# Autodesk Inventor assembly: CyberOrto
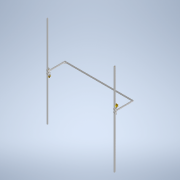
[picture p0: Inventor's stored thumbnail of the model, 180x180]
Saved by Autodesk Inventor 2022 (Build 260153000, 153)
## iProperties
RuleStatus: InUse
Created: 2021-12-29
Part Number: CyberOrto
Document SubType Name: Assembly
Designer: matte
Author: matte
## Documents named in this file (26)
- C:\Users\Elia\Documents\ELIA\UNITN\MAGISTRALE\1st year\1st semester\Mechanical Design\MDM-CyberOrto-CAD\CyberOrto.iam
- C:\Users\Elia\Documents\ELIA\UNITN\MAGISTRALE\1st year\1st semester\Mechanical Design\MDM-CyberOrto-CAD\Pezzi singoli\Trave Principale.ipt
- C:\Users\Elia\Documents\ELIA\UNITN\MAGISTRALE\1st year\1st semester\Mechanical Design\MDM-CyberOrto-CAD\Pezzi singoli\Supporto SX.ipt
- C:\Users\Elia\Documents\ELIA\UNITN\MAGISTRALE\1st year\1st semester\Mechanical Design\MDM-CyberOrto-CAD\Parker components\03-Brackets_Gussets_Plates\09-Machined Gussets\20-102.ipt
- C:\Users\Elia\Documents\ELIA\UNITN\MAGISTRALE\1st year\1st semester\Mechanical Design\MDM-CyberOrto-CAD\Parker components\02-Fasteners\10-Standard T-Nuts\20-050.ipt
- C:\Users\Elia\Documents\ELIA\UNITN\MAGISTRALE\1st year\1st semester\Mechanical Design\MDM-CyberOrto-CAD\Parker components\02-Fasteners\16-Screws\01-Metric Screws\01-Button Head\24-118-8.ipt
- C:\Users\Elia\Documents\ELIA\UNITN\MAGISTRALE\1st year\1st semester\Mechanical Design\MDM-CyberOrto-CAD\Guida a terra.iam
- C:\Users\Elia\Documents\ELIA\UNITN\MAGISTRALE\1st year\1st semester\Mechanical Design\MDM-CyberOrto-CAD\Parker components\05-Handles_Hinges\13-Pivot Joints\23-010.iam
- C:\Users\Elia\Documents\ELIA\UNITN\MAGISTRALE\1st year\1st semester\Mechanical Design\MDM-CyberOrto-CAD\Parker components\02-Fasteners\10-Standard T-Nuts\20-058.ipt
- C:\Users\Elia\Documents\ELIA\UNITN\MAGISTRALE\1st year\1st semester\Mechanical Design\MDM-CyberOrto-CAD\Parker components\02-Fasteners\16-Screws\01-Metric Screws\01-Button Head\24-116-8.ipt
- C:\Users\Elia\Documents\ELIA\UNITN\MAGISTRALE\1st year\1st semester\Mechanical Design\MDM-CyberOrto-CAD\Pezzi singoli\Supporto DX.ipt
- C:\Users\Elia\Documents\ELIA\UNITN\MAGISTRALE\1st year\1st semester\Mechanical Design\MDM-CyberOrto-CAD\Parker components\02-Fasteners\16-Screws\01-Metric Screws\01-Button Head\24-120-8.ipt
- C:\Users\Elia\Documents\ELIA\UNITN\MAGISTRALE\1st year\1st semester\Mechanical Design\MDM-CyberOrto-CAD\Pezzi singoli\Supporto lineare\Carrello semplice.iam
- C:\Users\Elia\Documents\ELIA\UNITN\MAGISTRALE\1st year\1st semester\Mechanical Design\MDM-CyberOrto-CAD\Platform.ipt
- C:\Users\Elia\Documents\ELIA\UNITN\MAGISTRALE\1st year\1st semester\Mechanical Design\MDM-CyberOrto-CAD\Parker components\02-Fasteners\16-Screws\01-Metric Screws\01-Button Head\24-130-6.ipt
- C:\Users\Elia\Documents\ELIA\UNITN\MAGISTRALE\1st year\1st semester\Mechanical Design\MDM-CyberOrto-CAD\Parker components\02-Fasteners\15-T-Bolts_Nuts_Washers\03-Washers\24-700-6.ipt
- C:\Users\Elia\Documents\ELIA\UNITN\MAGISTRALE\1st year\1st semester\Mechanical Design\MDM-CyberOrto-CAD\Parker components\02-Fasteners\15-T-Bolts_Nuts_Washers\02-Nuts\24-706-6.ipt
- C:\Users\Elia\Documents\ELIA\UNITN\MAGISTRALE\1st year\1st semester\Mechanical Design\MDM-CyberOrto-CAD\Servo Motor 50W\bch2mba531ca5c.ipt
- C:\Users\Elia\Documents\ELIA\UNITN\MAGISTRALE\1st year\1st semester\Mechanical Design\MDM-CyberOrto-CAD\Rack_Pinion\Rack gear scaled1.ipt
- C:\Users\Elia\Documents\ELIA\UNITN\MAGISTRALE\1st year\1st semester\Mechanical Design\MDM-CyberOrto-CAD\Rack_Pinion\pinion_scaled1.ipt
- C:\Users\Elia\Documents\ELIA\UNITN\MAGISTRALE\1st year\1st semester\Mechanical Design\MDM-CyberOrto-CAD\Inventor Support\Content Center Files\it-IT\ISO 1580\ISO 1580 - M4 x 12_.ipt
- C:\Users\Elia\Documents\ELIA\UNITN\MAGISTRALE\1st year\1st semester\Mechanical Design\MDM-CyberOrto-CAD\Inventor Support\Content Center Files\it-IT\AS 1474(1)\AS 1474 - M4(1).ipt
- C:\Users\Elia\Documents\ELIA\UNITN\MAGISTRALE\1st year\1st semester\Mechanical Design\MDM-CyberOrto-CAD\Trave a terra\Trave a terra.iam
- C:\Users\Elia\Documents\ELIA\UNITN\MAGISTRALE\1st year\1st semester\Mechanical Design\MDM-CyberOrto-CAD\Racks.iam
- C:\Users\Elia\Documents\ELIA\UNITN\MAGISTRALE\1st year\1st semester\Mechanical Design\MDM-CyberOrto-CAD\Parker components\02-Fasteners\16-Screws\01-Metric Screws\03-Socket Head\24-320-8SS.ipt
- C:\Users\Elia\Documents\ELIA\UNITN\MAGISTRALE\1st year\1st semester\Mechanical Design\MDM-CyberOrto-CAD\Parker components\02-Fasteners\10-Standard T-Nuts\20-058SS.ipt
## Components (86 placed, 25 different names)
1. Trave Principale:1 — Coincidente:1, Coincidente:2, Coincidente:3, Allineato:1, Coincidente:4, Allineato:2, Coincidente:5, Coincidente:10, Coincidente:40, Allineato:5, Allineato:6, Coincidente:41, Angolo:1
2. Supporto SX:1 — Allineato:1, Coincidente:4, Allineato:2, Coincidente:6, Allineato:3, Coincidente:7, Coincidente:15, Coincidente:16, Coincidente:23, Coincidente:28, Coincidente:29, Coincidente:30
3. Supporto DX:1 — Coincidente:45, Allineato:7, Allineato:8, Coincidente:48, Allineato:9, Allineato:10
4. Trave a terra:1 [sub-assembly] — Angolo:2, Angolo:3, Angolo:4, Allineato:59, Coincidente:130, Coincidente:169, Angolo:5, Coincidente:171, Allineato:62, Allineato:88, Coincidente:187, Coincidente:189
5. 20-058SS:1 — Coincidente:186, Coincidente:187
6. 20-058SS:2 — Coincidente:188, Coincidente:189
7. 24-118-8:3 — Coincidente:19, Coincidente:20
8. 24-118-8:4 — Coincidente:21, Coincidente:22
9. 20-050:2 — Coincidente:10, Coincidente:11, Coincidente:12
10. 24-118-8:1 — Coincidente:13, Coincidente:14
11. 24-118-8:2 — Coincidente:17, Coincidente:18
12. 20-102:1 — Coincidente:5, Coincidente:6, Allineato:3, Coincidente:8, Coincidente:9, Coincidente:11, Coincidente:12, Coincidente:13, Coincidente:14, Coincidente:17, Coincidente:18, Coincidente:19, Coincidente:20, Coincidente:21, Coincidente:22
13. 20-050:1 — Coincidente:7, Coincidente:8, Coincidente:9
14. 24-118-8:5 — Coincidente:31, Coincidente:32, Coincidente:33
15. 24-118-8:6 — Coincidente:34, Coincidente:35
16. 24-118-8:7 — Coincidente:38, Coincidente:39
17. 24-118-8:8 — Coincidente:36, Coincidente:37
18. Guida a terra:1 [sub-assembly] — Coincidente:15, Coincidente:16, Coincidente:23, Coincidente:32, Coincidente:33, Coincidente:34, Coincidente:35, Coincidente:36, Coincidente:37, Coincidente:38, Coincidente:39, Coincidente:138, Coincidente:139, Allineato:61, Coincidente:141, Coincidente:143, Coincidente:145, Coincidente:162
19. 20-050:3 — Coincidente:27, Allineato:4, Coincidente:28, Coincidente:30, Coincidente:31
20. 20-050:4 — Coincidente:27, Allineato:4, Coincidente:29
21. 23-010:1 [sub-assembly] — Coincidente:40, Allineato:5, Allineato:6, Coincidente:43, Coincidente:44, Coincidente:45, Allineato:7, Allineato:8, Coincidente:46, Coincidente:47
22. 20-058:1 — Coincidente:41, Angolo:1, Coincidente:42
23. 24-116-8:1 — Coincidente:42, Coincidente:43, Coincidente:44
24. 24-120-8:1 — Coincidente:46, Coincidente:47
25. 24-120-8:2 — Coincidente:51, Coincidente:52
26. Carrello semplice:1 [sub-assembly] — Coincidente:48, Allineato:9, Allineato:10, Coincidente:51, Coincidente:52, Coincidente:53, Allineato:13, Coincidente:54, Coincidente:56, Coincidente:58, Coincidente:60, Coincidente:62, Angolo:2, Angolo:3, Angolo:4, Allineato:59, Coincidente:130
27. 24-130-6:1 — Inserimento:1, Coincidente:61
28. 24-700-6:1 — Inserimento:1, Inserimento:7
29. 24-706-6:1 — Coincidente:55, Coincidente:56
30. 24-130-6:2 — Coincidente:59
31. 24-700-6:3 — Inserimento:6
32. 24-130-6:3 — Coincidente:57
33. 24-700-6:2 — Inserimento:8
34. 24-130-6:4 — Coincidente:55
35. 24-700-6:4 — Inserimento:5
36. 24-706-6:2 — Coincidente:57, Coincidente:58
37. 24-706-6:3 — Coincidente:61, Coincidente:62
38. 24-706-6:4 — Coincidente:59, Coincidente:60
39. Platform:1 — Coincidente:53, Allineato:13, Coincidente:54, Inserimento:5, Inserimento:6, Inserimento:7, Inserimento:8, Coincidente:63, Coincidente:64, Coincidente:65, Coincidente:66, Coincidente:67, Coincidente:68, Coincidente:114, Coincidente:117, Coincidente:121, Coincidente:125, Coincidente:129
40. ISO 1580 M4 x 12:2 — Coincidente:126, Coincidente:127, Coincidente:128
41. AS 1474 - Metrico M4:2 — Coincidente:120, Coincidente:121
42. AS 1474 - Metrico M4:3 — Coincidente:124, Coincidente:125
43. AS 1474 - Metrico M4:4 — Coincidente:128, Coincidente:129
44. ISO 1580 M4 x 12:4 — Coincidente:118, Coincidente:119, Coincidente:120
45. ISO 1580 M4 x 12:3 — Coincidente:122, Coincidente:123, Coincidente:124
46. AS 1474 - Metrico M4:1 — Coincidente:116, Coincidente:117
47. ISO 1580 M4 x 12:1 — Coincidente:114, Coincidente:115, Coincidente:116
48. bch2mba531ca5c:1 — Coincidente:66, Coincidente:67, Coincidente:68, Coincidente:113, Coincidente:115, Coincidente:118, Coincidente:119, Coincidente:122, Coincidente:123, Coincidente:126, Coincidente:127
49. pinion_scaled1:1 — Coincidente:113, Tangente:1, Allineato:87
50. 24-706-6:8 — Coincidente:142, Coincidente:143
51. 24-706-6:7 — Coincidente:140, Coincidente:141
52. 24-706-6:6 — Coincidente:144, Coincidente:145
53. 24-700-6:8
54. 24-130-6:8 — Coincidente:146
55. 24-700-6:7
56. 24-130-6:7 — Coincidente:144
57. 24-700-6:6
58. 24-706-6:5 — Coincidente:146, Coincidente:162
59. 24-700-6:5
60. Platform:3 — Coincidente:138, Coincidente:139, Allineato:61, Coincidente:158, Coincidente:159, Coincidente:160, Coincidente:164, Coincidente:166, Coincidente:167, Coincidente:168
61. 24-130-6:5 — Coincidente:142
62. 24-130-6:6 — Coincidente:140
63. bch2mba531ca5c:2 — Coincidente:158, Coincidente:161
64. ISO 1580 M4 x 12:5 — Coincidente:161
65. AS 1474 - Metrico M4:5 — Coincidente:167
66. ISO 1580 M4 x 12:6 — Coincidente:159, Coincidente:163
67. AS 1474 - Metrico M4:6 — Coincidente:168
68. AS 1474 - Metrico M4:7 — Coincidente:165, Coincidente:166
69. ISO 1580 M4 x 12:7 — Coincidente:165
70. AS 1474 - Metrico M4:8 — Coincidente:163, Coincidente:164
71. ISO 1580 M4 x 12:8 — Coincidente:160
72. Racks:5 [sub-assembly] — Allineato:73, Allineato:74, Coincidente:177, Allineato:75, Allineato:76, Coincidente:178
73. Racks:6 [sub-assembly] — Allineato:75, Allineato:76, Coincidente:178, Coincidente:180, Allineato:77, Allineato:78
74. Racks:7 [sub-assembly] — Coincidente:180, Allineato:77, Allineato:78, Allineato:79, Allineato:80, Coincidente:181
75. Racks:8 [sub-assembly] — Allineato:79, Allineato:80, Coincidente:181, Coincidente:182, Allineato:81, Allineato:82
76. Racks:9 [sub-assembly] — Coincidente:182, Allineato:81, Allineato:82, Allineato:85, Allineato:86, Coincidente:185
77. Rack gear scaled1:2 — Allineato:85, Allineato:86, Coincidente:185
78. 24-320-8SS:3
79. 24-320-8SS:4 — Coincidente:188
80. Racks:4 [sub-assembly] — Coincidente:174, Allineato:67, Allineato:68, Allineato:69, Allineato:70, Coincidente:175
81. Racks:3 [sub-assembly] — Allineato:71, Coincidente:176, Allineato:72, Allineato:73, Allineato:74, Coincidente:177
82. Racks:2 [sub-assembly] — Allineato:69, Allineato:70, Coincidente:175, Allineato:71, Coincidente:176, Allineato:72
83. Rack gear scaled1:1 — Coincidente:170, Coincidente:171, Allineato:62, Allineato:63, Allineato:64, Coincidente:172, Allineato:65, Coincidente:173, Allineato:66
84. 24-320-8SS:1 — Coincidente:172, Allineato:65, Coincidente:186
85. 24-320-8SS:2 — Coincidente:173, Allineato:66
86. Racks:1 [sub-assembly] — Coincidente:169, Angolo:5, Coincidente:170, Allineato:63, Allineato:64, Coincidente:174, Allineato:67, Allineato:68, Allineato:87, Allineato:88
## Relationships (192: Mate 130, Flush 40, Insert 16, Angle 5, Tangent 1)
- Coincidente:1 [Mate]: Trave Principale:1
- Coincidente:2 [Mate]: Trave Principale:1
- Coincidente:3 [Mate]: Trave Principale:1
- Allineato:1 [Flush]: Trave Principale:1 ↔ Supporto SX:1
- Coincidente:4 [Mate]: Trave Principale:1 ↔ Supporto SX:1
- Allineato:2 [Flush]: Trave Principale:1 ↔ Supporto SX:1
- Coincidente:5 [Mate]: Trave Principale:1 ↔ 20-102:1
- Coincidente:6 [Mate]: Supporto SX:1 ↔ 20-102:1
- Allineato:3 [Flush]: Supporto SX:1 ↔ 20-102:1
- Coincidente:7 [Mate]: Supporto SX:1 ↔ 20-050:1
- Coincidente:8 [Mate]: 20-102:1 ↔ 20-050:1
- Coincidente:9 [Mate]: 20-102:1 ↔ 20-050:1
- Coincidente:10 [Mate]: Trave Principale:1 ↔ 20-050:2
- Coincidente:11 [Mate]: 20-050:2 ↔ 20-102:1
- Coincidente:12 [Mate]: 20-050:2 ↔ 20-102:1
- Coincidente:13 [Mate]: 24-118-8:1 ↔ 20-102:1
- Coincidente:14 [Mate]: 24-118-8:1 ↔ 20-102:1
- Coincidente:15 [Mate]: Supporto SX:1 ↔ Guida a terra:1
- Coincidente:16 [Mate]: Supporto SX:1 ↔ Guida a terra:1
- Coincidente:17 [Mate]: 24-118-8:2 ↔ 20-102:1
- Coincidente:18 [Mate]: 24-118-8:2 ↔ 20-102:1
- Coincidente:19 [Mate]: 24-118-8:3 ↔ 20-102:1
- Coincidente:20 [Mate]: 24-118-8:3 ↔ 20-102:1
- Coincidente:21 [Mate]: 24-118-8:4 ↔ 20-102:1
- Coincidente:22 [Mate]: 24-118-8:4 ↔ 20-102:1
- Coincidente:23 [Mate]: Supporto SX:1 ↔ Guida a terra:1
- Coincidente:27 [Mate]: 20-050:3 ↔ 20-050:4
- Allineato:4 [Flush]: 20-050:3 ↔ 20-050:4
- Coincidente:28 [Mate]: Supporto SX:1 ↔ 20-050:3
- Coincidente:29 [Mate]: Supporto SX:1 ↔ 20-050:4
- Coincidente:30 [Mate]: Supporto SX:1 ↔ 20-050:3
- Coincidente:31 [Mate]: 24-118-8:5 ↔ 20-050:3
- Coincidente:32 [Mate]: 24-118-8:5 ↔ Guida a terra:1
- Coincidente:33 [Mate]: 24-118-8:5 ↔ Guida a terra:1
- Coincidente:34 [Mate]: 24-118-8:6 ↔ Guida a terra:1
- Coincidente:35 [Mate]: 24-118-8:6 ↔ Guida a terra:1
- Coincidente:36 [Mate]: 24-118-8:8 ↔ Guida a terra:1
- Coincidente:37 [Mate]: 24-118-8:8 ↔ Guida a terra:1
- Coincidente:38 [Mate]: 24-118-8:7 ↔ Guida a terra:1
- Coincidente:39 [Mate]: 24-118-8:7 ↔ Guida a terra:1
- Coincidente:40 [Mate]: Trave Principale:1 ↔ 23-010:1
- Allineato:5 [Flush]: Trave Principale:1 ↔ 23-010:1
- Allineato:6 [Flush]: Trave Principale:1 ↔ 23-010:1
- Coincidente:41 [Mate]: Trave Principale:1 ↔ 20-058:1
- Angolo:1 [Angle] (0 deg): Trave Principale:1 ↔ 20-058:1
- Coincidente:42 [Mate]: 20-058:1 ↔ 24-116-8:1
- Coincidente:43 [Mate]: 23-010:1 ↔ 24-116-8:1
- Coincidente:44 [Mate]: 23-010:1 ↔ 24-116-8:1
- Coincidente:45 [Mate]: Supporto DX:1 ↔ 23-010:1
- Allineato:7 [Flush]: Supporto DX:1 ↔ 23-010:1
- Allineato:8 [Flush]: Supporto DX:1 ↔ 23-010:1
- Coincidente:46 [Mate]: 23-010:1 ↔ 24-120-8:1
- Coincidente:47 [Mate]: 23-010:1 ↔ 24-120-8:1
- Coincidente:48 [Mate]: Supporto DX:1 ↔ Carrello semplice:1
- Allineato:9 [Flush]: Supporto DX:1 ↔ Carrello semplice:1
- Allineato:10 [Flush]: Supporto DX:1 ↔ Carrello semplice:1
- Coincidente:51 [Mate]: 24-120-8:2 ↔ Carrello semplice:1
- Coincidente:52 [Mate]: 24-120-8:2 ↔ Carrello semplice:1
- Coincidente:53 [Mate]: Carrello semplice:1 ↔ Platform:1
- Allineato:13 [Flush]: Carrello semplice:1 ↔ Platform:1
- Coincidente:54 [Mate]: Carrello semplice:1 ↔ Platform:1
- Inserimento:1: 24-130-6:1 ↔ 24-700-6:1
- [Insert]: 24-130-6:2 ↔ 24-700-6:2
- [Insert]: 24-700-6:3 ↔ 24-130-6:3
- [Insert]: 24-130-6:4 ↔ 24-700-6:4
- Inserimento:5: 24-700-6:4 ↔ Platform:1
- Inserimento:6: 24-700-6:3 ↔ Platform:1
- Inserimento:7: 24-700-6:1 ↔ Platform:1
- Inserimento:8: 24-700-6:2 ↔ Platform:1
- Coincidente:55 [Mate]: 24-706-6:1 ↔ 24-130-6:4
- Coincidente:56 [Mate]: Carrello semplice:1 ↔ 24-706-6:1
- Coincidente:57 [Mate]: 24-130-6:3 ↔ 24-706-6:2
- Coincidente:58 [Mate]: Carrello semplice:1 ↔ 24-706-6:2
- Coincidente:59 [Mate]: 24-130-6:2 ↔ 24-706-6:4
- Coincidente:60 [Mate]: Carrello semplice:1 ↔ 24-706-6:4
- Coincidente:61 [Mate]: 24-130-6:1 ↔ 24-706-6:3
- Coincidente:62 [Mate]: Carrello semplice:1 ↔ 24-706-6:3
- Coincidente:63 [Mate]: Platform:1
- Coincidente:64 [Mate]: Platform:1
- Coincidente:65 [Mate]: Platform:1
- Coincidente:66 [Mate]: Platform:1 ↔ bch2mba531ca5c:1
- Coincidente:67 [Mate]: Platform:1 ↔ bch2mba531ca5c:1
- Coincidente:68 [Mate]: Platform:1 ↔ bch2mba531ca5c:1
- Coincidente:113 [Mate]: bch2mba531ca5c:1 ↔ pinion_scaled1:1
- Tangente:1: pinion_scaled1:1
- Coincidente:114 [Mate]: Platform:1 ↔ ISO 1580 M4 x 12:1
- Coincidente:115 [Mate]: ISO 1580 M4 x 12:1 ↔ bch2mba531ca5c:1
- Coincidente:116 [Mate]: AS 1474 - Metrico M4:1 ↔ ISO 1580 M4 x 12:1
- Coincidente:117 [Mate]: Platform:1 ↔ AS 1474 - Metrico M4:1
- Coincidente:118 [Mate]: ISO 1580 M4 x 12:4 ↔ bch2mba531ca5c:1
- Coincidente:119 [Mate]: ISO 1580 M4 x 12:4 ↔ bch2mba531ca5c:1
- Coincidente:120 [Mate]: AS 1474 - Metrico M4:2 ↔ ISO 1580 M4 x 12:4
- Coincidente:121 [Mate]: Platform:1 ↔ AS 1474 - Metrico M4:2
- Coincidente:122 [Mate]: ISO 1580 M4 x 12:3 ↔ bch2mba531ca5c:1
- Coincidente:123 [Mate]: ISO 1580 M4 x 12:3 ↔ bch2mba531ca5c:1
- Coincidente:124 [Mate]: AS 1474 - Metrico M4:3 ↔ ISO 1580 M4 x 12:3
- Coincidente:125 [Mate]: Platform:1 ↔ AS 1474 - Metrico M4:3
- Coincidente:126 [Mate]: ISO 1580 M4 x 12:2 ↔ bch2mba531ca5c:1
- Coincidente:127 [Mate]: ISO 1580 M4 x 12:2 ↔ bch2mba531ca5c:1
- Coincidente:128 [Mate]: ISO 1580 M4 x 12:2 ↔ AS 1474 - Metrico M4:4
- Coincidente:129 [Mate]: Platform:1 ↔ AS 1474 - Metrico M4:4
- Angolo:2 [Angle] (0 deg): Trave a terra:1 ↔ Carrello semplice:1
- Angolo:3 [Angle] (0 deg): Trave a terra:1 ↔ Carrello semplice:1
- Angolo:4 [Angle] (0 deg): Trave a terra:1 ↔ Carrello semplice:1
- Allineato:59 [Flush] (19 mm): Trave a terra:1 ↔ Carrello semplice:1
- Coincidente:130 [Mate] (20 mm): Trave a terra:1 ↔ Carrello semplice:1
- [Insert]: 24-700-6:5 ↔ 24-130-6:5
- [Insert]: 24-700-6:6 ↔ 24-130-6:6
- [Insert]: 24-700-6:7 ↔ 24-130-6:7
- [Insert]: 24-700-6:8 ↔ 24-130-6:8
- [Insert]: 24-700-6:8 ↔ Platform:3
- [Insert]: 24-700-6:7 ↔ Platform:3
- [Insert]: 24-700-6:5 ↔ Platform:3
- [Insert]: 24-700-6:6 ↔ Platform:3
- Coincidente:138 [Mate]: Guida a terra:1 ↔ Platform:3
- Coincidente:139 [Mate]: Guida a terra:1 ↔ Platform:3
- Allineato:61 [Flush]: Guida a terra:1 ↔ Platform:3
- Coincidente:140 [Mate]: 24-706-6:7 ↔ 24-130-6:6
- Coincidente:141 [Mate]: Guida a terra:1 ↔ 24-706-6:7
- Coincidente:142 [Mate]: 24-706-6:8 ↔ 24-130-6:5
- Coincidente:143 [Mate]: Guida a terra:1 ↔ 24-706-6:8
- Coincidente:144 [Mate]: 24-706-6:6 ↔ 24-130-6:7
- Coincidente:145 [Mate]: Guida a terra:1 ↔ 24-706-6:6
- Coincidente:146 [Mate]: 24-130-6:8 ↔ 24-706-6:5
- [Mate]: bch2mba531ca5c:2 ↔ ISO 1580 M4 x 12:5
- [Mate]: ISO 1580 M4 x 12:5 ↔ AS 1474 - Metrico M4:5
- [Mate]: bch2mba531ca5c:2 ↔ ISO 1580 M4 x 12:8
- [Mate]: bch2mba531ca5c:2 ↔ ISO 1580 M4 x 12:8
- [Mate]: AS 1474 - Metrico M4:6 ↔ ISO 1580 M4 x 12:8
- [Mate]: bch2mba531ca5c:2 ↔ ISO 1580 M4 x 12:7
- [Mate]: bch2mba531ca5c:2 ↔ ISO 1580 M4 x 12:7
- [Mate]: bch2mba531ca5c:2 ↔ ISO 1580 M4 x 12:6
- [Mate]: bch2mba531ca5c:2 ↔ ISO 1580 M4 x 12:6
- Coincidente:158 [Mate]: Platform:3 ↔ bch2mba531ca5c:2
- Coincidente:159 [Mate]: Platform:3 ↔ ISO 1580 M4 x 12:6
- Coincidente:160 [Mate]: Platform:3 ↔ ISO 1580 M4 x 12:8
- Coincidente:161 [Mate]: bch2mba531ca5c:2 ↔ ISO 1580 M4 x 12:5
- Coincidente:162 [Mate]: Guida a terra:1 ↔ 24-706-6:5
- Coincidente:163 [Mate]: ISO 1580 M4 x 12:6 ↔ AS 1474 - Metrico M4:8
- Coincidente:164 [Mate]: Platform:3 ↔ AS 1474 - Metrico M4:8
- Coincidente:165 [Mate]: AS 1474 - Metrico M4:7 ↔ ISO 1580 M4 x 12:7
- Coincidente:166 [Mate]: Platform:3 ↔ AS 1474 - Metrico M4:7
- Coincidente:167 [Mate]: Platform:3 ↔ AS 1474 - Metrico M4:5
- Coincidente:168 [Mate]: Platform:3 ↔ AS 1474 - Metrico M4:6
- Coincidente:169 [Mate]: Trave a terra:1 ↔ Racks:1
- Angolo:5 [Angle] (0 deg): Trave a terra:1 ↔ Racks:1
- Coincidente:170 [Mate]: Rack gear scaled1:1 ↔ Racks:1
- Coincidente:171 [Mate]: Trave a terra:1 ↔ Rack gear scaled1:1
- Allineato:62 [Flush]: Trave a terra:1 ↔ Rack gear scaled1:1
- Allineato:63 [Flush]: Rack gear scaled1:1 ↔ Racks:1
- Allineato:64 [Flush]: Rack gear scaled1:1 ↔ Racks:1
- Coincidente:172 [Mate]: Rack gear scaled1:1 ↔ 24-320-8SS:1
- Allineato:65 [Flush]: Rack gear scaled1:1 ↔ 24-320-8SS:1
- Coincidente:173 [Mate]: Rack gear scaled1:1 ↔ 24-320-8SS:2
- Allineato:66 [Flush]: Rack gear scaled1:1 ↔ 24-320-8SS:2
- Coincidente:174 [Mate]: Racks:4 ↔ Racks:1
- Allineato:67 [Flush]: Racks:4 ↔ Racks:1
- Allineato:68 [Flush]: Racks:4 ↔ Racks:1
- Allineato:69 [Flush]: Racks:4 ↔ Racks:2
- Allineato:70 [Flush]: Racks:4 ↔ Racks:2
- Coincidente:175 [Mate]: Racks:4 ↔ Racks:2
- Allineato:71 [Flush]: Racks:3 ↔ Racks:2
- Coincidente:176 [Mate]: Racks:3 ↔ Racks:2
- Allineato:72 [Flush]: Racks:3 ↔ Racks:2
- Allineato:73 [Flush]: Racks:5 ↔ Racks:3
- Allineato:74 [Flush]: Racks:5 ↔ Racks:3
- Coincidente:177 [Mate]: Racks:5 ↔ Racks:3
- Allineato:75 [Flush]: Racks:5 ↔ Racks:6
- Allineato:76 [Flush]: Racks:5 ↔ Racks:6
- Coincidente:178 [Mate]: Racks:5 ↔ Racks:6
- Coincidente:180 [Mate]: Racks:6 ↔ Racks:7
- Allineato:77 [Flush]: Racks:6 ↔ Racks:7
- Allineato:78 [Flush]: Racks:6 ↔ Racks:7
- Allineato:79 [Flush]: Racks:7 ↔ Racks:8
- Allineato:80 [Flush]: Racks:7 ↔ Racks:8
- Coincidente:181 [Mate]: Racks:7 ↔ Racks:8
- Coincidente:182 [Mate]: Racks:8 ↔ Racks:9
- Allineato:81 [Flush]: Racks:8 ↔ Racks:9
- Allineato:82 [Flush]: Racks:8 ↔ Racks:9
- [Mate]: Rack gear scaled1:2 ↔ 24-320-8SS:3
- [Flush]: Rack gear scaled1:2 ↔ 24-320-8SS:3
- [Mate]: Rack gear scaled1:2 ↔ 24-320-8SS:4
- [Flush]: Rack gear scaled1:2 ↔ 24-320-8SS:4
- Allineato:85 [Flush]: Racks:9 ↔ Rack gear scaled1:2
- Allineato:86 [Flush]: Racks:9 ↔ Rack gear scaled1:2
- Coincidente:185 [Mate]: Racks:9 ↔ Rack gear scaled1:2
- Allineato:87 [Flush]: pinion_scaled1:1 ↔ Racks:1
- Allineato:88 [Flush] (-13 mm): Trave a terra:1 ↔ Racks:1
- Coincidente:186 [Mate]: 20-058SS:1 ↔ 24-320-8SS:1
- Coincidente:187 [Mate]: Trave a terra:1 ↔ 20-058SS:1
- Coincidente:188 [Mate]: 20-058SS:2 ↔ 24-320-8SS:4
- Coincidente:189 [Mate]: Trave a terra:1 ↔ 20-058SS:2
## Named parameters: L_piatto_guide = 240 mm, L_tracce_terra = 4000 mm, L_traccia_superiore = 3000 mm, H_supporto = 700 mm, d116_d115 = 0 mm, d117_d115 = 0 mm, d118_d115 = 0 mm, d311_d115 = 0 mm, d312_d116_d115 = 0 mm, d313_d117_d115 = 0 mm, d314_d118_d115 = 0 mm, d315_d119 = 0 mm, d316_d120 = 0 mm, d317_d121 = 0 mm, d318_d122 = 0 mm, d333_d234 = 0 mm, d334_d235 = 0 mm, d335_d237 = 0 mm, d336_d238 = 0 mm, d337_d239 = 0 mm, d338_d241 = 0 mm, d339_d242 = 0 mm, d341_d245 = 0 mm, d342_d246 = 0 mm, d398_d369 = 0 mm, d399_d370 = 0 mm, d400_d371 = 0 mm, d401_d372 = 0 mm
